# Autodesk Inventor assembly: VP-Dual-BAG
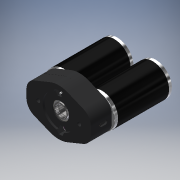
[picture p0: Inventor's stored thumbnail of the model, 180x180]
Saved by Autodesk Inventor 2019 (Build 230136000, 136)
## iProperties
Created: 2018-08-19
Part Number: VP-Dual-BAG
Document SubType Name: Assembly
Designer: Rafi
Author: Rafi
## Documents named in this file (15)
- C:\Users\Rafi Pedersen\Documents\GrabCAD\Common Parts Library\Gearboxes\Planetary Gearboxes\V2 Stages\Dual Input Stage\VP Dual BAG Input.iam
- C:\Users\Rafi Pedersen\Documents\GrabCAD\Common Parts Library\Gearboxes\Planetary Gearboxes\V2 Stages\Dual Input Housing.ipt
- C:\Users\Rafi Pedersen\Documents\GrabCAD\Common Parts Library\Shaft Accessories\Bearings\Bearing\17mm ID x 26mm OD x 5mm WD Radial Bearing.ipt
- C:\Users\Rafi Pedersen\Documents\GrabCAD\Common Parts Library\Shaft Accessories\Bearings\Bearing.ipt
- C:\Users\Rafi Pedersen\Documents\GrabCAD\Common Parts Library\Gearboxes\Planetary Gearboxes\V2 Stages\Dual Input Alignment Pin.ipt
- C:\Users\Rafi Pedersen\Documents\GrabCAD\Common Parts Library\Gearboxes\Planetary Gearboxes\Screws\8-32 Lock Nut.ipt
- C:\Users\Rafi Pedersen\Documents\GrabCAD\Common Parts Library\Gearboxes\Planetary Gearboxes\Screws\8-32 x 0.75in Screw.ipt
- C:\Users\Rafi Pedersen\Documents\GrabCAD\Common Parts Library\Gearboxes\Planetary Gearboxes\Screws\M4 x 10mm Screw.ipt
- C:\Users\Rafi Pedersen\Documents\GrabCAD\Common Parts Library\Gearboxes\Planetary Gearboxes\V2 Stages\Dual Input Output Gear.ipt
- C:\Users\Rafi Pedersen\Documents\GrabCAD\Common Parts Library\Gearboxes\Planetary Gearboxes\V2 Stages\Dual Input Coupler Gear.ipt
- C:\Users\Rafi Pedersen\Documents\GrabCAD\Common Parts Library\Gearboxes\Planetary Gearboxes\Input Coupler\Coupler Set Screw.ipt
- C:\Users\Rafi Pedersen\Documents\GrabCAD\Common Parts Library\Motors\BAG.ipt
- C:\Users\Rafi Pedersen\Documents\GrabCAD\Common Parts Library\Gearboxes\Planetary Gearboxes\V2 Stages\BAG Dual Input.ipt
- C:\Users\Rafi Pedersen\Documents\GrabCAD\Common Parts Library\Gearboxes\Planetary Gearboxes\Input Coupler\4mm Coupler Sleeve.ipt
- C:\Users\Rafi Pedersen\Documents\GrabCAD\Common Parts Library\Gearboxes\Planetary Gearboxes\V2 Stages\Dual Input Stage.iam
## Components (22 placed, 12 different names)
1. Dual Input Housing:1 — Insert:1, Insert:3, Insert:4, Angle:1, Insert:5, Angle:2, Mate:3, Mate:8, Mate:9, Mate:10, Mate:11
2. 17mm ID x 26mm OD x 5mm WD Radial Bearing:1 — Insert:1, Insert:15
3. 17mm ID x 26mm OD x 5mm WD Radial Bearing:2 — Insert:35
4. Dual Input Alignment Pin:1 — Insert:3
5. 8-32 Lock Nut:1 — Insert:4, Angle:1
6. 8-32 Lock Nut:2 — Insert:5, Angle:2
7. 8-32 x 0.75in Screw:1 — Flush:1, Mate:8, Mate:12
8. 8-32 x 0.75in Screw:2 — Mate:3, Flush:1
9. M4 x 10mm Screw:1 — Insert:31
10. M4 x 10mm Screw:2 — Insert:34
11. M4 x 10mm Screw:3 — Insert:32
12. M4 x 10mm Screw:4 — Insert:33
13. Dual Input Output Gear:1 — Insert:15, Rotation:1, Rotation:2
14. Dual Input Coupler Gear:1 — Rotation:2, Mate:5, Tangent:2, Insert:27, Flush:2, Angle:5
15. Dual Input Coupler Gear:2 — Rotation:1, Mate:4, Tangent:1, Insert:28, Flush:2, Angle:6
16. Coupler Set Screw:1 — Mate:4, Tangent:1
17. Coupler Set Screw:2 — Mate:5, Tangent:2
18. BAG:1 — Insert:26, Insert:29, Mate:13
19. BAG:2 — Insert:25, Insert:30, Mate:14
20. 4mm Coupler Sleeve:1 — Insert:25, Insert:27, Angle:5
21. 4mm Coupler Sleeve:2 — Insert:26, Insert:28, Angle:6
22. BAG Dual Input:1 — Mate:9, Mate:10, Mate:11, Mate:12, Insert:29, Insert:30, Mate:13, Mate:14, Insert:31, Insert:32, Insert:33, Insert:34, Insert:35
## Relationships (36: Insert 16, Mate 10, Angle 4, Flush 2, RelateRotation 2, Tangent 2)
- Insert:1: Dual Input Housing:1 ↔ 17mm ID x 26mm OD x 5mm WD Radial Bearing:1
- Insert:3: Dual Input Housing:1 ↔ Dual Input Alignment Pin:1
- Insert:4: Dual Input Housing:1 ↔ 8-32 Lock Nut:1
- Angle:1 (0 deg): Dual Input Housing:1 ↔ 8-32 Lock Nut:1
- Insert:5: Dual Input Housing:1 ↔ 8-32 Lock Nut:2
- Angle:2 (0 deg): Dual Input Housing:1 ↔ 8-32 Lock Nut:2
- Mate:3: Dual Input Housing:1 ↔ 8-32 x 0.75in Screw:2
- Flush:1: 8-32 x 0.75in Screw:1 ↔ 8-32 x 0.75in Screw:2
- Insert:15: 17mm ID x 26mm OD x 5mm WD Radial Bearing:1 ↔ Dual Input Output Gear:1
- Rotation:1 [RelateRotation] (1 ul): Dual Input Output Gear:1 ↔ Dual Input Coupler Gear:2
- Rotation:2 [RelateRotation] (1 ul): Dual Input Output Gear:1 ↔ Dual Input Coupler Gear:1
- Mate:4: Dual Input Coupler Gear:2 ↔ Coupler Set Screw:1
- Tangent:1: Dual Input Coupler Gear:2 ↔ Coupler Set Screw:1
- Mate:5: Dual Input Coupler Gear:1 ↔ Coupler Set Screw:2
- Tangent:2: Dual Input Coupler Gear:1 ↔ Coupler Set Screw:2
- Insert:25: BAG:2 ↔ 4mm Coupler Sleeve:1
- Insert:26: BAG:1 ↔ 4mm Coupler Sleeve:2
- Insert:27: Dual Input Coupler Gear:1 ↔ 4mm Coupler Sleeve:1
- Insert:28: Dual Input Coupler Gear:2 ↔ 4mm Coupler Sleeve:2
- Mate:8: Dual Input Housing:1 ↔ 8-32 x 0.75in Screw:1
- Mate:9: Dual Input Housing:1 ↔ BAG Dual Input:1
- Mate:10: Dual Input Housing:1 ↔ BAG Dual Input:1
- Mate:11: Dual Input Housing:1 ↔ BAG Dual Input:1
- Mate:12: 8-32 x 0.75in Screw:1 ↔ BAG Dual Input:1
- Flush:2: Dual Input Coupler Gear:1 ↔ Dual Input Coupler Gear:2
- Insert:29: BAG:1 ↔ BAG Dual Input:1
- Insert:30: BAG:2 ↔ BAG Dual Input:1
- Mate:13: BAG:1 ↔ BAG Dual Input:1
- Mate:14: BAG:2 ↔ BAG Dual Input:1
- Insert:31: M4 x 10mm Screw:1 ↔ BAG Dual Input:1
- Insert:32: M4 x 10mm Screw:3 ↔ BAG Dual Input:1
- Insert:33: M4 x 10mm Screw:4 ↔ BAG Dual Input:1
- Insert:34: M4 x 10mm Screw:2 ↔ BAG Dual Input:1
- Insert:35: 17mm ID x 26mm OD x 5mm WD Radial Bearing:2 ↔ BAG Dual Input:1
- Angle:5 (0 deg): Dual Input Coupler Gear:1 ↔ 4mm Coupler Sleeve:1
- Angle:6 (0 deg): Dual Input Coupler Gear:2 ↔ 4mm Coupler Sleeve:2
